# Autodesk Inventor assembly: Twitter
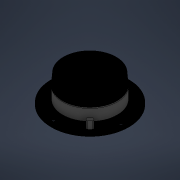
[picture p0: Inventor's stored thumbnail of the model, 180x180]
Saved by Autodesk Inventor 2022 (Build 260153070, 153G)
## iProperties
Created: 2021-11-19
Part Number: Twitter
Document SubType Name: Assembly
Designer: kalugin_a
Author: kalugin_a
## Documents named in this file (6)
- C:\Users\kalugin_a\Documents\Inventor\TUTO\MELAS\Workspace\Twitter.iam
- C:\Users\kalugin_a\Documents\Inventor\TUTO\MELAS\Workspace\Фланец.ipt
- C:\Users\kalugin_a\Documents\Inventor\TUTO\MELAS\Workspace\Clemm.ipt
- C:\Users\kalugin_a\Documents\Inventor\TUTO\MELAS\Workspace\Magnetic.ipt
- C:\Users\kalugin_a\Documents\Inventor\TUTO\MELAS\Workspace\DOME.ipt
- C:\Users\kalugin_a\Documents\Inventor\TUTO\MELAS\Workspace\CUP.ipt
## Components (8 placed, 5 different names)
1. Фланец:1 — Жесткий:1, Заподлицо:1
2. Magnetic:1 — Заподлицо:1
3. DOME:1
4. CUP:1
5. Clemm:1 — Жесткий:1
6. Clemm:2
7. Clemm:3
8. Clemm:4
## Component patterns: (4 elements, first: Clemm:1)
## Relationships (2: WeldJoint 1, Flush 1)
- Жесткий:1 [WeldJoint]: Фланец:1 ↔ Clemm:1
- Заподлицо:1 [Flush]: Фланец:1 ↔ Magnetic:1
